# Autodesk Inventor assembly: Soporte_motor_encoder
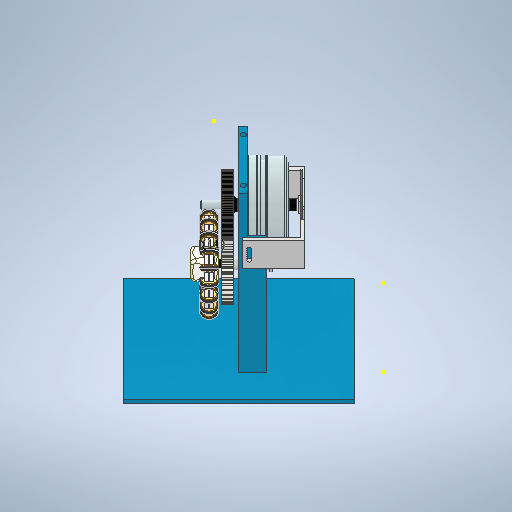
[picture p0: Inventor's stored thumbnail of the model, 512x512]
Saved by Autodesk Inventor 2025.1 (Build 291241000, 241)
## iProperties
Created: 2025-10-26
Part Number: Soporte_motor_encoder
Document SubType Name: Assembly
Designer: paeze
Author: paeze
## Documents named in this file (10)
- J:\URUBOTS\Base_Ruedas\28_08\Soporte_motor_encoder.iam
- J:\URUBOTS\Base_Ruedas\28_08\Soporte motor para encoder.ipt
- J:\URUBOTS\Base_Ruedas\387266-ec45fl-30w-a-kabel\387266_ec45fl_30w_a_kabel\387266_ec45fl_30w_a_kabel\387266_ec45fl_30w_a_kabel.ipt
- J:\URUBOTS\Base_Ruedas\gtf-robots-50mm-omniwheel-1.snapshot.2\GTF Robots 50mm Wheel v4\GTF Robots 50mm Wheel v4\GTF Robots 50mm Wheel v4.ipt
- J:\URUBOTS\Base_Ruedas\Eje.ipt
- J:\URUBOTS\Base_Ruedas\28_08\Ruleman.ipt
- J:\URUBOTS\Base_Ruedas\28_08\EngranajeChico.ipt
- J:\URUBOTS\Base_Ruedas\28_08\EngranajeGrande.ipt
- J:\URUBOTS\Base_Ruedas\28_08\Encoder.ipt
- J:\URUBOTS\Base_Ruedas\28_08\Soporte encoder.ipt
## Components (9 placed, 9 different names)
1. Soporte motor para encoder:1 — Rigid:1, Rigid:2
2. 387266_ec45fl_30w_a_kabel:1 — Rigid:1, Rigid:3, Rotational:1
3. GTF Robots 50mm Wheel v4:1 — Rigid:6
4. Eje:1 — Rigid:4, Rigid:5, Rigid:6
5. Ruleman:1 — Rigid:2, Rigid:4
6. Spur Gear1:1 — Rigid:3
7. Spur Gear2:1 — Rigid:5
8. Encoder:1 — Rotational:1, Rigid:7
9. Soporte encoder:1 — Rigid:7
## Relationships (8: WeldJoint 7, RevoluteJoint 1)
- Rigid:1 [WeldJoint]: Soporte motor para encoder:1 ↔ 387266_ec45fl_30w_a_kabel:1
- Rigid:2 [WeldJoint]: Soporte motor para encoder:1 ↔ Ruleman:1
- Rigid:3 [WeldJoint] (8 mm): 387266_ec45fl_30w_a_kabel:1 ↔ Spur Gear1:1
- Rigid:4 [WeldJoint] (-6 mm): Eje:1 ↔ Ruleman:1
- Rigid:5 [WeldJoint] (-3.2 mm): Eje:1 ↔ Spur Gear2:1
- Rigid:6 [WeldJoint] (-5 mm): GTF Robots 50mm Wheel v4:1 ↔ Eje:1
- Rotational:1 [RevoluteJoint] (1 mm): 387266_ec45fl_30w_a_kabel:1 ↔ Encoder:1
- Rigid:7 [WeldJoint]: Encoder:1 ↔ Soporte encoder:1
